# Autodesk Inventor assembly: AnsambluSpinner
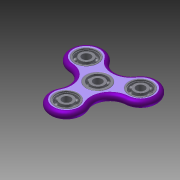
[picture p0: Inventor's stored thumbnail of the model, 180x180]
Saved by Autodesk Inventor 2011 SP2 (Build 150309200, 309)
## iProperties
Created: 2023-02-27
Part Number: AnsambluSpinner
Document SubType Name: Assembly
Designer: utilizator
Author: utilizator
## Documents named in this file (6)
- D:\Studenti\Donisan Enya 1322b\AnsambluSpinner.iam
- D:\Studenti\Donisan Enya 1322b\FidgetSpinnerBody.ipt
- D:\Studenti\Donisan Enya 1322b\AnsambluSpinner\Design Accelerator\Bearing1.iam
- D:\Studenti\Donisan Enya 1322b\AnsambluSpinner\Design Accelerator\Bearing2.iam
- D:\Studenti\Donisan Enya 1322b\AnsambluSpinner\Design Accelerator\Bearing3.iam
- D:\Studenti\Donisan Enya 1322b\AnsambluSpinner\Design Accelerator\Bearing4.iam
## Components (5 placed, 2 different names)
1. FidgetSpinnerBody:1 — Mate:1, Mate:2, Mate:3, Mate:4, Mate:5, Mate:6, Mate:7, Mate:8, Mate:9, Mate:10, Mate:11, Angle:1
2. Bearing:1 [sub-assembly] — Mate:1, Mate:2, Mate:5
3. Bearing:2 [sub-assembly] — Mate:6, Mate:7
4. Bearing:3 [sub-assembly] — Mate:8, Mate:9
5. Bearing:4 [sub-assembly] — Mate:10, Mate:11
## Relationships (12: Mate 11, Angle 1)
- Mate:1: FidgetSpinnerBody:1 ↔ Bearing:1
- Mate:2: FidgetSpinnerBody:1 ↔ Bearing:1
- Mate:3: FidgetSpinnerBody:1
- Mate:4: FidgetSpinnerBody:1
- Mate:5: FidgetSpinnerBody:1 ↔ Bearing:1
- Mate:6: FidgetSpinnerBody:1 ↔ Bearing:2
- Mate:7: FidgetSpinnerBody:1 ↔ Bearing:2
- Mate:8: FidgetSpinnerBody:1 ↔ Bearing:3
- Mate:9: FidgetSpinnerBody:1 ↔ Bearing:3
- Mate:10: FidgetSpinnerBody:1 ↔ Bearing:4
- Mate:11: FidgetSpinnerBody:1 ↔ Bearing:4
- Angle:1 (0 deg): FidgetSpinnerBody:1
